# Autodesk Inventor assembly: nsysm1810502dp
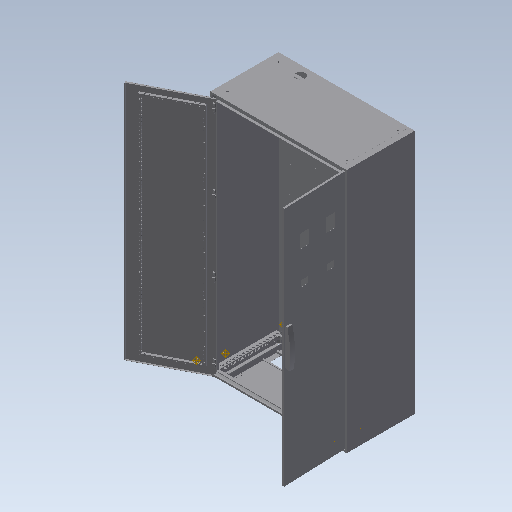
[picture p0: Inventor's stored thumbnail of the model, 512x512]
Saved by Autodesk Inventor 2021 (Build 250183000, 183)
## iProperties
Company: TraceParts S.A.
Created: 2018-06-25
Part Number: nsysm1810502dp
Checked By: TraceParts S.A.
Catalog Web Link: www.traceparts.com
Document SubType Name: Assembly
Designer: TraceParts
REFERENCE: NSYSM1810502DP
DESIGN: Compact metal enclosures Spacial SM with mounting plate, 1800x1000x500, 2 door(s)
SUPPLIER: Schneider Electric
TraceParts.PartNumber: 10-28052009-086210
TraceParts.PartTitle: Compact metal enclosures Spacial SM with mounting plate
TraceParts.InstanceId: 10-28052009-086210IH6OUMLYN3HEZGFA4RR094XI
TraceParts.PartStatus: Published
TraceParts.PartVersion: 1.2.7
TRACEPARTS: TRACEPARTS
TraceParts.PartLanguage: en
TraceParts.ClassPath: SCHNEIDER_ELECTRIC_DISTRI:/SCHNEIDER_DISTRI/F_SCHNEIDER_ELECTRIC_ENVEL/SCHNEIDER_ELECTRIC_ENVEL.120/SCHNEIDER_ELECTRIC_ENVEL.120.010/SCHNEIDER_ELECTRIC_ENVEL.120.010.030/SCHNEIDER_ELECTRIC_ENVEL.120.010.030.010/10-28052009-086210
Author: TraceParts
## Documents named in this file (7)
- C:\Users\andre\Documents\GitHub\Dis.-Mecatronico-E6\inventor proyecto\Tablero\Armario\nsysm1810502dp.iam
- C:\Users\andre\Documents\GitHub\Dis.-Mecatronico-E6\inventor proyecto\Tablero\Armario\nsysm1810502dp_01.ipt
- C:\Users\andre\Documents\GitHub\Dis.-Mecatronico-E6\inventor proyecto\Tablero\Armario\nsysm1810502dp_02.ipt
- C:\Users\andre\Documents\GitHub\Dis.-Mecatronico-E6\inventor proyecto\Tablero\Armario\nsysm1810502dp_03.ipt
- C:\Users\andre\Documents\GitHub\Dis.-Mecatronico-E6\inventor proyecto\Tablero\Armario\nsysm1810502dp_04.ipt
- C:\Users\andre\Documents\GitHub\Dis.-Mecatronico-E6\inventor proyecto\Tablero\Armario\nsysm1810502dp_05.ipt
- C:\Users\andre\Documents\GitHub\Dis.-Mecatronico-E6\inventor proyecto\Tablero\Armario\nsysm1810502dp_06.ipt
## Components (6 placed, 6 different names)
1. nsysm1810502dp_01:1 — Rotational:1, Rotational:2
2. nsysm1810502dp_02:1
3. nsysm1810502dp_03:1
4. nsysm1810502dp_04:1 — Rotational:2
5. nsysm1810502dp_05:1 — Rotational:1
6. nsysm1810502dp_06:1
## Relationships (2: RevoluteJoint 2)
- Rotational:1 [RevoluteJoint]: nsysm1810502dp_01:1 ↔ nsysm1810502dp_05:1
- Rotational:2 [RevoluteJoint]: nsysm1810502dp_01:1 ↔ nsysm1810502dp_04:1
